# Autodesk Inventor assembly: Total
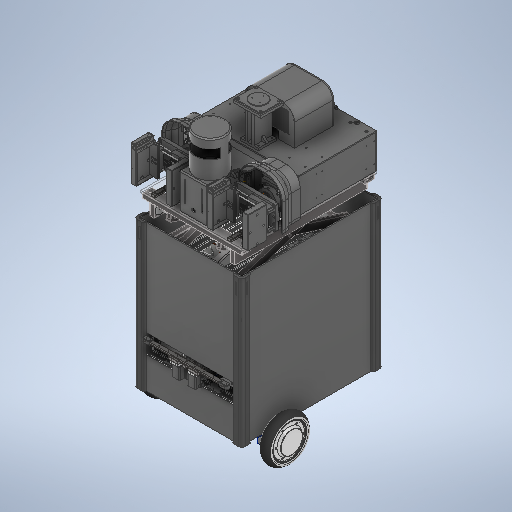
[picture p0: Inventor's stored thumbnail of the model, 512x512]
Saved by Autodesk Inventor 2026.2 (Build 302298010, 298A)
## iProperties
Created: 2026-05-16
Part Number: Total
Document SubType Name: Assembly
Designer: chris
Author: chris
## Documents named in this file (4)
- C:\Users\chanh\내 드라이브\교과공부\2026년 1학기 (4학년 1학기)\01창의제품설계\UMMA_CAD\01완성품\Total.iam
- C:\Users\chanh\내 드라이브\교과공부\2026년 1학기 (4학년 1학기)\01창의제품설계\UMMA_CAD\02하체\02하체.iam
- C:\Users\chanh\내 드라이브\교과공부\2026년 1학기 (4학년 1학기)\01창의제품설계\UMMA_CAD\03상체\2nd floor.iam
- C:\Users\chanh\내 드라이브\교과공부\2026년 1학기 (4학년 1학기)\01창의제품설계\UMMA_CAD\04그리퍼\3rd_floor.iam
## Components (3 placed, 3 different names)
1. 02하체:1 [sub-assembly] — Flush:1, Flush:2, Flush:3, Mate:1, Flush:4, Mate:2, Mate:4, Mate:5
2. 2nd floor:1 [sub-assembly] — Mate:1, Flush:4, Mate:2, Mate:3
3. 3rd_floor:1 [sub-assembly] — Mate:3, Mate:4, Mate:5
## Relationships (9: Mate 5, Flush 4)
- Flush:1: 02하체:1
- Flush:2: 02하체:1
- Flush:3: 02하체:1
- Mate:1: 02하체:1 ↔ 2nd floor:1
- Flush:4: 02하체:1 ↔ 2nd floor:1
- Mate:2: 02하체:1 ↔ 2nd floor:1
- Mate:3: 2nd floor:1 ↔ 3rd_floor:1
- Mate:4: 02하체:1 ↔ 3rd_floor:1
- Mate:5: 02하체:1 ↔ 3rd_floor:1
